# Autodesk Inventor assembly: MasterAssembly
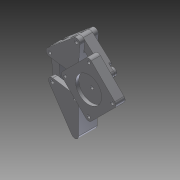
[picture p0: Inventor's stored thumbnail of the model, 180x180]
Saved by Autodesk Inventor 2011 SP2 (Build 150309200, 309)
## iProperties
Created: 2014-05-08
Part Number: MasterAssembly
Document SubType Name: Assembly
Designer: Maurice Woods
Author: Maurice Woods
## Documents named in this file (8)
- C:\Users\Maurice\Documents\GitHub\strandbeest\MasterAssembly.iam
- C:\Users\Maurice\Documents\GitHub\strandbeest\BDE.ipt
- C:\Users\Maurice\Documents\GitHub\strandbeest\GHI.ipt
- C:\Users\Maurice\Documents\Github\strandbeest\F.ipt
- C:\Users\Maurice\Documents\GitHub\strandbeest\C.ipt
- C:\Users\Maurice\Documents\GitHub\strandbeest\J.ipt
- C:\Users\Maurice\Documents\GitHub\strandbeest\K.ipt
- C:\Users\Maurice\Documents\GitHub\strandbeest\MatingPlates.ipt
## Components (7 placed, 7 different names)
1. BDE:1 — Mate:2, Flush:3, Mate:3, Mate:10, Mate:11, Mate:13
2. GHI:1 — Flush:1, Mate:4, Mate:5, Mate:6, Mate:12
3. F:1 — Flush:2, Mate:3, Mate:4
4. C:1 — Mate:2, Flush:4, Mate:5, Mate:6
5. J:1 — Flush:5, Mate:13, Mate:14
6. K:1 — Flush:6, Mate:12, Mate:14
7. MatingPlates:1 — Mate:10, Mate:11
## Relationships (16: Mate 10, Flush 6)
- Flush:1: GHI:1
- Flush:2: F:1
- Mate:2: BDE:1 ↔ C:1
- Flush:3: BDE:1
- Flush:4: C:1
- Flush:5: J:1
- Flush:6: K:1
- Mate:3: BDE:1 ↔ F:1
- Mate:4: GHI:1 ↔ F:1
- Mate:5: GHI:1 ↔ C:1
- Mate:6: GHI:1 ↔ C:1
- Mate:10: BDE:1 ↔ MatingPlates:1
- Mate:11: BDE:1 ↔ MatingPlates:1
- Mate:12: GHI:1 ↔ K:1
- Mate:13: BDE:1 ↔ J:1
- Mate:14: J:1 ↔ K:1
## Named parameters: ScaleFactor = 1, LengthA = 25.4 mm, LengthB = 27.73947 mm, LengthC = 26.26896 mm, LengthD = 26.80368 mm, LengthE = 37.29789 mm, LengthF = 26.33579 mm, LengthG = 24.53104 mm, LengthH = 43.91525 mm, LengthI = 32.75254 mm, LengthJ = 33.42104 mm, LengthK = 41.37525 mm, LengthL = 5.21368 mm, LengthM = 10.02632 mm
